# Autodesk Inventor assembly: lower
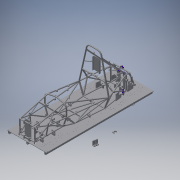
[picture p0: Inventor's stored thumbnail of the model, 180x180]
Saved by Autodesk Inventor 2018.2 (Build 222227000, 227)
## iProperties
Company: none
Created: 2018-05-02
Part Number: lower
Material: 一般
Description: CATIA V5 STEP Exchange
Document SubType Name: Assembly
Designer: ku_sk
Authority: none
Title: C:\Users\formula\Dropbox\共有ファイル(桑野)\lower.stp
Author: none
Sending System: CATIA V5 STEP AP203
Preprocessor: CATIA Version 5 Release 17 (IN-10)
## Documents named in this file (12)
- C:\Users\ku_sk\Documents\Inventor\Aero\KS-15\裏付け資料\lower.iam
- C:\Users\ku_sk\Documents\Inventor\Aero\KS-15\裏付け資料\jouban.ipt
- C:\Users\ku_sk\Documents\Inventor\Aero\KS-15\裏付け資料\karikuni14a.ipt
- C:\Users\ku_sk\Documents\Inventor\Aero\KS-15\裏付け資料\fai26 alminium jig.ipt
- C:\Users\ku_sk\Documents\Inventor\Aero\KS-15\裏付け資料\fai29 alminium jig.ipt
- C:\Users\ku_sk\Documents\Inventor\Aero\KS-15\裏付け資料\ike-ru syou ana.ipt
- C:\Users\ku_sk\Documents\Inventor\Aero\KS-15\裏付け資料\jigu1(67-55.7-20).ipt
- C:\Users\ku_sk\Documents\Inventor\Aero\KS-15\裏付け資料\front bulkhead jigu.ipt
- C:\Users\ku_sk\Documents\Inventor\Aero\KS-15\裏付け資料\main hoop brace support lower.ipt
- C:\Users\ku_sk\Documents\Inventor\Aero\KS-15\裏付け資料\rear lower.ipt
- C:\Users\ku_sk\Documents\Inventor\Aero\KS-15\Fr.wing\parts\stay\Bracket.ipt
- C:\Users\ku_sk\Documents\Inventor\Aero\KS-15\Fr.wing\parts\stay\Bracket1.ipt
## Components (50 placed, 50 different names)
1. Bracket:1 — メイト:1, メイト:2, メイト:3
2. Bracket1:1 — メイト:4, メイト:5
3. jouban.1
4. karikuni11a.1 — メイト:1, メイト:2, メイト:3, メイト:4, メイト:5
5. fai26 alminium jig.1
6. fai29 alminium jig.1
7. ike-ru syou ana.1
8. jigu1(67-55.7-20).1
9. jigu1(67-55.7-20).2
10. fai26 alminium jig.2
11. jigu1(67-55.7-20).3
12. fai26 alminium jig.3
13. fai26 alminium jig.4
14. jigu1(67-55.7-20).4
15. jigu1(67-55.7-20).5
16. fai26 alminium jig.5
17. jigu1(67-55.7-20).6
18. fai26 alminium jig.6
19. jigu1(67-55.7-20).7
20. fai26 alminium jig.7
21. jigu1(67-55.7-20).8
22. fai26 alminium jig.8
23. front bulkhead jigu
24. fai26 alminium jig.9
25. fai26 alminium jig.10
26. fai26 alminium jig.11
27. fai26 alminium jig.12
28. fai26 alminium jig.13
29. fai26 alminium jig.14
30. fai26 alminium jig.15
31. fai26 alminium jig.16
32. fai26 alminium jig.17
33. fai26 alminium jig.18
34. fai26 alminium jig.19
35. fai26 alminium jig.20
36. main hoop brace support lower
37. fai26 alminium jig.21
38. main hoop brace support lower.1
39. rear lower
40. fai26 alminium jig.22
41. rear lower.1
42. fai26 alminium jig.23
43. jigu1(67-55.7-20).9
44. fai26 alminium jig.24
45. jigu1(67-55.7-20).10
46. fai26 alminium jig.25
47. jigu1(67-55.7-20).11
48. fai26 alminium jig.26
49. jigu1(67-55.7-20).12
50. fai26 alminium jig.27
## Relationships (5: Mate 5)
- メイト:1 [Mate]: Bracket:1 ↔ karikuni11a.1
- メイト:2 [Mate]: Bracket:1 ↔ karikuni11a.1
- メイト:3 [Mate]: Bracket:1 ↔ karikuni11a.1
- メイト:4 [Mate]: Bracket1:1 ↔ karikuni11a.1
- メイト:5 [Mate]: Bracket1:1 ↔ karikuni11a.1
